# Autodesk Inventor assembly: Fretboard
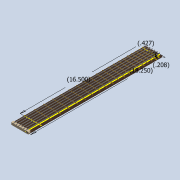
[picture p0: Inventor's stored thumbnail of the model, 180x180]
Saved by Autodesk Inventor 2021 (Build 250183000, 183)
## iProperties
Created: 2021-03-17
Part Number: Fretboard
Document SubType Name: Assembly
Designer: Tom
Author: Tom
## Documents named in this file (5)
- C:\Users\Tom\Documents\Inventor\Guitar\Fretboard.iam
- C:\Users\Tom\Documents\Inventor\Guitar\Base_for_Frets.ipt
- C:\Users\Tom\Documents\Inventor\Guitar\Fret.ipt
- C:\Users\Tom\Documents\Inventor\Guitar\String.ipt
- C:\Users\Tom\Documents\Inventor\Guitar\Nut.ipt
## Components (28 placed, 4 different names)
1. Base_for_Frets:1 — Mate:1, Flush:1, Flush:2, Mate:2, Flush:3, Flush:4, Mate:3, Flush:5, Flush:6, Mate:4, Flush:7, Flush:8, Mate:5, Flush:9, Flush:10, Mate:6, Flush:11, Flush:12, Mate:7, Flush:13, Flush:14, Mate:8, Flush:15, Flush:16, Mate:9, Flush:17, Flush:18, Mate:10, Flush:19, Flush:20, Mate:11, Flush:21, Flush:22, Mate:12, Flush:23, Flush:24, Mate:13, Flush:25, Flush:26, Mate:14, Flush:27, Flush:28, Mate:15, Flush:29, Flush:30, Mate:16, Flush:31, Flush:32, Mate:17, Flush:33, Flush:34, Mate:18, Flush:35, Flush:36, Mate:19, Flush:37, Flush:38, Mate:20, Flush:39, Flush:40, Flush:42, Mate:21, Flush:43, Flush:44
2. Fret:1 — Mate:1, Flush:1, Flush:2
3. Fret:2 — Mate:2, Flush:3, Flush:4
4. Fret:3 — Mate:3, Flush:5, Flush:6
5. Fret:4 — Mate:4, Flush:7, Flush:8
6. Fret:5 — Mate:5, Flush:9, Flush:10
7. Fret:6 — Mate:6, Flush:11, Flush:12
8. Fret:7 — Mate:7, Flush:13, Flush:14
9. Fret:8 — Mate:8, Flush:15, Flush:16
10. Fret:9 — Mate:9, Flush:17, Flush:18
11. Fret:10 — Mate:10, Flush:19, Flush:20
12. Fret:11 — Mate:11, Flush:21, Flush:22
13. Fret:12 — Mate:12, Flush:23, Flush:24
14. Fret:13 — Mate:13, Flush:25, Flush:26
15. Fret:14 — Mate:14, Flush:27, Flush:28
16. Fret:15 — Mate:15, Flush:29, Flush:30
17. Fret:16 — Mate:16, Flush:31, Flush:32
18. Fret:17 — Mate:17, Flush:33, Flush:34
19. Fret:18 — Mate:18, Flush:35, Flush:36
20. Fret:19 — Mate:19, Flush:37, Flush:38
21. Fret:20 — Mate:20, Flush:39, Flush:40
22. Nut:1 — Mate:21, Flush:43, Flush:44, Flush:41
23. String:1 — Flush:41, Flush:42
24. String:2
25. String:3
26. String:4
27. String:5
28. String:6
## Component patterns: (6 elements, first: String:1)
## Relationships (65: Flush 44, Mate 21)
- Mate:1: Base_for_Frets:1 ↔ Fret:1
- Flush:1: Base_for_Frets:1 ↔ Fret:1
- Flush:2 (37.3062 mm): Base_for_Frets:1 ↔ Fret:1
- Mate:2: Base_for_Frets:1 ↔ Fret:2
- Flush:3: Base_for_Frets:1 ↔ Fret:2
- Flush:4 (72.2313 mm): Base_for_Frets:1 ↔ Fret:2
- Mate:3: Base_for_Frets:1 ↔ Fret:3
- Flush:5: Base_for_Frets:1 ↔ Fret:3
- Flush:6 (104.2458 mm): Base_for_Frets:1 ↔ Fret:3
- Mate:4: Base_for_Frets:1 ↔ Fret:4
- Flush:7: Base_for_Frets:1 ↔ Fret:4
- Flush:8 (135.4667 mm): Base_for_Frets:1 ↔ Fret:4
- Mate:5: Base_for_Frets:1 ↔ Fret:5
- Flush:9: Base_for_Frets:1 ↔ Fret:5
- Flush:10 (163.5125 mm): Base_for_Frets:1 ↔ Fret:5
- Mate:6: Base_for_Frets:1 ↔ Fret:6
- Flush:11: Base_for_Frets:1 ↔ Fret:6
- Flush:12 (191.2937 mm): Base_for_Frets:1 ↔ Fret:6
- Mate:7: Base_for_Frets:1 ↔ Fret:7
- Flush:13: Base_for_Frets:1 ↔ Fret:7
- Flush:14 (216.6937 mm): Base_for_Frets:1 ↔ Fret:7
- Mate:8: Base_for_Frets:1 ↔ Fret:8
- Flush:15: Base_for_Frets:1 ↔ Fret:8
- Flush:16 (241.3 mm): Base_for_Frets:1 ↔ Fret:8
- Mate:9: Base_for_Frets:1 ↔ Fret:9
- Flush:17: Base_for_Frets:1 ↔ Fret:9
- Flush:18 (264.0542 mm): Base_for_Frets:1 ↔ Fret:9
- Mate:10: Base_for_Frets:1 ↔ Fret:10
- Flush:19: Base_for_Frets:1 ↔ Fret:10
- Flush:20 (286.2792 mm): Base_for_Frets:1 ↔ Fret:10
- Mate:11: Base_for_Frets:1 ↔ Fret:11
- Flush:21: Base_for_Frets:1 ↔ Fret:11
- Flush:22 (306.9167 mm): Base_for_Frets:1 ↔ Fret:11
- Mate:12: Base_for_Frets:1 ↔ Fret:12
- Flush:23: Base_for_Frets:1 ↔ Fret:12
- Flush:24 (326.2313 mm): Base_for_Frets:1 ↔ Fret:12
- Mate:13: Base_for_Frets:1 ↔ Fret:13
- Flush:25: Base_for_Frets:1 ↔ Fret:13
- Flush:26 (344.4875 mm): Base_for_Frets:1 ↔ Fret:13
- Mate:14: Base_for_Frets:1 ↔ Fret:14
- Flush:27: Base_for_Frets:1 ↔ Fret:14
- Flush:28 (361.95 mm): Base_for_Frets:1 ↔ Fret:14
- Mate:15: Base_for_Frets:1 ↔ Fret:15
- Flush:29: Base_for_Frets:1 ↔ Fret:15
- Flush:30 (377.825 mm): Base_for_Frets:1 ↔ Fret:15
- Mate:16: Base_for_Frets:1 ↔ Fret:16
- Flush:31: Base_for_Frets:1 ↔ Fret:16
- Flush:32 (393.7 mm): Base_for_Frets:1 ↔ Fret:16
- Mate:17: Base_for_Frets:1 ↔ Fret:17
- Flush:33: Base_for_Frets:1 ↔ Fret:17
- Flush:34 (407.1938 mm): Base_for_Frets:1 ↔ Fret:17
- Mate:18: Base_for_Frets:1 ↔ Fret:18
- Flush:35: Base_for_Frets:1 ↔ Fret:18
- Flush:36 (420.6875 mm): Base_for_Frets:1 ↔ Fret:18
- Mate:19: Base_for_Frets:1 ↔ Fret:19
- Flush:37: Base_for_Frets:1 ↔ Fret:19
- Flush:38 (433.3875 mm): Base_for_Frets:1 ↔ Fret:19
- Mate:20: Base_for_Frets:1 ↔ Fret:20
- Flush:39: Base_for_Frets:1 ↔ Fret:20
- Flush:40 (445.5583 mm): Base_for_Frets:1 ↔ Fret:20
- Flush:41: Nut:1 ↔ String:1
- Flush:42 (8.3911 mm): Base_for_Frets:1 ↔ String:1
- Mate:21: Base_for_Frets:1 ↔ Nut:1
- Flush:43: Base_for_Frets:1 ↔ Nut:1
- Flush:44: Base_for_Frets:1 ↔ Nut:1
